# Autodesk Inventor assembly: Assembly1
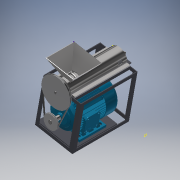
[picture p0: Inventor's stored thumbnail of the model, 180x180]
Saved by Autodesk Inventor 2019 (Build 230136000, 136)
## iProperties
Created: 2017-11-11
Part Number: Assembly1
Document SubType Name: Assembly
Designer: Mr.Duc
Author: Mr.Duc
## Documents named in this file (13)
- C:\Users\Usuario\Desktop\8vo semestre\comunitarias\diseño\Assembly1.iam
- C:\Users\Usuario\Desktop\8vo semestre\comunitarias\diseño\nap sau.ipt
- C:\Users\Usuario\Desktop\8vo semestre\comunitarias\diseño\than.ipt
- C:\Users\Mr.Duc\Documents\Inventor\Content Center Files\R2018\en-US\ISO 7046-1(1)\DIN EN ISO 7046-1 - M8 x 14 - 4.8 - H.ipt
- E:\Inventor 2017\VHD INVENTOR\DACTM\DONG CO\Assembly1\Design Accelerator\Bearing1.iam
- C:\Users\Usuario\Desktop\8vo semestre\comunitarias\diseño\truc.ipt
- C:\Users\Usuario\Desktop\8vo semestre\comunitarias\diseño\nap truoc.ipt
- C:\Users\Mr.Duc\Documents\Inventor\Content Center Files\R2018\en-US\BS EN ISO 4016\BS EN ISO 4016 - M10x65.ipt
- C:\Users\Mr.Duc\Documents\Inventor\Content Center Files\R2018\en-US\ISO 4032(2)\ISO 4032 - M10 - ISO.ipt
- E:\Inventor 2017\VHD INVENTOR\DACTM\DONG CO\long soc.ipt
- C:\Users\Usuario\Desktop\8vo semestre\comunitarias\diseño\Ensamblaje1.iam
- C:\Users\Usuario\Desktop\8vo semestre\comunitarias\diseño\Assembly1\Design Accelerator\Transmisión de correa trapezoidal1.iam
- C:\Users\Usuario\Desktop\8vo semestre\comunitarias\diseño\Assembly1\Design Accelerator\Rodamiento1.iam
## Components (22 placed, 12 different names)
1. nap sau:1 — Mate:1, Mate:2, Mate:3, Mate:4, Mate:6, Mate:7
2. than:1 — Mate:1, Mate:2, Mate:8, Mate:9, Mate:10, Mate:11, Mate:12, Flush:2, Mate:14, Mate:16, Mate:17, Mate:18, Insert:2, Flush:3, Coincidencia:20
3. DIN EN ISO 7046-1 H M8 x 14 - 4.8 - H:4 — Mate:3, Mate:10
4. DIN EN ISO 7046-1 H M8 x 14 - 4.8 - H:2 — Mate:4, Mate:9
5. DIN EN ISO 7046-1 H M8 x 14 - 4.8 - H:3 — Mate:6, Mate:11
6. DIN EN ISO 7046-1 H M8 x 14 - 4.8 - H:1 — Mate:7, Mate:8
7. Bearing:1 [sub-assembly] — Mate:12, Flush:2, Mate:13
8. truc:1 — Mate:13, Mate:14, Mate:15, Nivelación:5, Coincidencia:19
9. nap truoc:1 — Mate:15, Mate:16, Mate:17, Mate:18, Insert:1
10. long soc:1 — Flush:3
11. Ensamblaje1:1 [sub-assembly] — Nivelación:5, Coincidencia:19, Coincidencia:20, Coincidencia:21, Coincidencia:22, Coincidencia:23
12. Transmisión de correa trapezoidal:1 [sub-assembly]
13. Rodamiento:1 [sub-assembly] — Coincidencia:21, Coincidencia:22
14. Rodamiento:2 [sub-assembly] — Coincidencia:23
15. BS EN ISO 4016 M10x65:1 — Insert:1
16. BS EN ISO 4016 M10x65:2
17. BS EN ISO 4016 M10x65:3
18. BS EN ISO 4016 M10x65:4
19. ISO 4032 M10:1 — Insert:2
20. ISO 4032 M10:2
21. ISO 4032 M10:3
22. ISO 4032 M10:4
## Component patterns: (4 elements, first: BS EN ISO 4016 M10x65:1), (4 elements, first: ISO 4032 M10:1)
## Relationships (27: Mate 22, Flush 3, Insert 2)
- Mate:1: nap sau:1 ↔ than:1
- Mate:2: nap sau:1 ↔ than:1
- Mate:3: nap sau:1 ↔ DIN EN ISO 7046-1 H M8 x 14 - 4.8 - H:4
- Mate:4: nap sau:1 ↔ DIN EN ISO 7046-1 H M8 x 14 - 4.8 - H:2
- Mate:6: nap sau:1 ↔ DIN EN ISO 7046-1 H M8 x 14 - 4.8 - H:3
- Mate:7: nap sau:1 ↔ DIN EN ISO 7046-1 H M8 x 14 - 4.8 - H:1
- Mate:8 (0.5 mm): than:1 ↔ DIN EN ISO 7046-1 H M8 x 14 - 4.8 - H:1
- Mate:9 (0.5 mm): than:1 ↔ DIN EN ISO 7046-1 H M8 x 14 - 4.8 - H:2
- Mate:10 (0.5 mm): than:1 ↔ DIN EN ISO 7046-1 H M8 x 14 - 4.8 - H:4
- Mate:11 (0.5 mm): than:1 ↔ DIN EN ISO 7046-1 H M8 x 14 - 4.8 - H:3
- Mate:12: than:1 ↔ Bearing:1
- Flush:2: than:1 ↔ Bearing:1
- Mate:13: Bearing:1 ↔ truc:1
- Mate:14: than:1 ↔ truc:1
- Mate:15: truc:1 ↔ nap truoc:1
- Mate:16: than:1 ↔ nap truoc:1
- Mate:17: than:1 ↔ nap truoc:1
- Mate:18: than:1 ↔ nap truoc:1
- Insert:1: nap truoc:1 ↔ BS EN ISO 4016 M10x65:1
- Insert:2: than:1 ↔ ISO 4032 M10:1
- Flush:3: than:1 ↔ long soc:1
- Nivelación:5 [Flush]: truc:1 ↔ Ensamblaje1:1
- Coincidencia:19 [Mate] (324 mm): truc:1 ↔ Ensamblaje1:1
- Coincidencia:20 [Mate]: than:1 ↔ Ensamblaje1:1
- Coincidencia:21 [Mate]: Ensamblaje1:1 ↔ Rodamiento:1
- Coincidencia:22 [Mate]: Ensamblaje1:1 ↔ Rodamiento:1
- Coincidencia:23 [Mate]: Ensamblaje1:1 ↔ Rodamiento:2
